# Autodesk Inventor assembly: Drive Roller Assembly
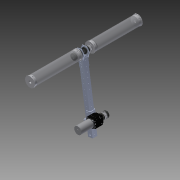
[picture p0: Inventor's stored thumbnail of the model, 180x180]
Saved by Autodesk Inventor 2014 SP1 (Build 180222100, 222)
## iProperties
Created: 2014-01-12
Part Number: Drive Roller Assembly
Document SubType Name: Assembly
Designer: Michael
Mass: 1125.53 g
Surface Area: 3756.72 cm^2
Volume: 516.176 cm^3
Density: 2.18052 g/cm^3
Author: Michael
## Documents named in this file (17)
- C:\Users\Arpan\Documents\GitHub\2014buildCAD\Collector\Drive Roller Assembly.iam
- C:\Users\Arpan\Documents\GitHub\2014buildCAD\Collector\Hex Shaft Collar 1-2 in (7552K500).ipt
- C:\Users\Arpan\Documents\GitHub\2014buildCAD\Collector\Timing Pulley (HTD 5mm) - 18T 9mm Double Flange, 1-2 in Hex (VexPro).ipt
- C:\Users\Arpan\Documents\GitHub\2014buildCAD\Collector\Hex Bearing 1-2 in (FR8ZZ-Hex, am-0279).ipt
- C:\Users\Arpan\Documents\GitHub\2014buildCAD\Collector\Hex Shaft 1-2 in (am-0856).ipt
- C:\Users\Arpan\Documents\GitHub\2014buildCAD\Collector\Roller End Cap Drive (3-D Printed).ipt
- C:\Users\Arpan\Documents\GitHub\2014buildCAD\Funnel Catcher\Vex Pro End Bearing Mount.ipt
- C:\Users\Arpan\Documents\GitHub\2014buildCAD\Funnel Catcher\Vex Pro 1x1 rectangular tubing 14 in length.ipt
- C:\Users\Arpan\Documents\GitHub\2014buildCAD\Collector\VersaPlanetary.iam
- C:\Users\Arpan\Documents\GitHub\2014buildCAD\Collector\Vex Pro VersaPlanetary Side Mount.ipt
- C:\Users\Arpan\Documents\GitHub\2014buildCAD\Collector\Polycarbonate Roller 2 OD 1-16 Thick (8585K64).ipt
- C:\Users\Arpan\Documents\GitHub\2014buildCAD\Collector\Drive Roller Assembly\AIP\FEA\axi0epmtc.fins
- C:\Users\Arpan\Documents\GitHub\2014buildCAD\Collector\Drive Roller Assembly\AIP\FEA\axi0epmu8.fsat
- C:\Users\Arpan\Documents\GitHub\2014buildCAD\Collector\Drive Roller Assembly\AIP\FEA\axi0epmu8.ftes
- C:\Users\Arpan\Documents\GitHub\2014buildCAD\Collector\Drive Roller Assembly\AIP\FEA\axi0epmu8.fwiz
- C:\Users\Arpan\Documents\GitHub\2014buildCAD\Collector\Drive Roller Assembly\AIP\FEA\axi0epnk0.fmsh
- C:\Users\Arpan\Documents\GitHub\2014buildCAD\Collector\Drive Roller Assembly\AIP\FEA\axi0epoao.fres
## Components (19 placed, 10 different names)
1. Timing Pulley (HTD 5mm) - 18T 9mm Double Flange, 1-2 in Hex (VexPro):1 — Mate:25, Mate:26, Mate:49, Mate:50
2. Hex Bearing 1-2 in (FR8ZZ-Hex, am-0279):1 — Insert:8, Mate:55, Mate:56, Mate:57
3. Hex Shaft Collar 1-2 in (7552K500):5 — Mate:31, Mate:32, Mate:50, Mate:55
4. Hex Shaft 1-2 in (am-0856):1 — Mate:25, Mate:26, Mate:31, Mate:32, Mate:33, Mate:34, Flush:1, Mate:56, Mate:57, Mate:59, Mate:60, Mate:62, Mate:63, Mate:84, Mate:85, Mate:88, Mate:89, Mate:91, Mate:92
5. Roller End Cap Drive (3-D Printed):1 — Mate:33, Mate:34, Flush:1, Mate:49, Insert:25, Mate:86, Mate:90
6. Vex Pro End Bearing Mount:1 — Insert:8, Mate:58, Insert:15, Insert:16
7. Hex Bearing 1-2 in (FR8ZZ-Hex, am-0279):2 — Insert:9, Mate:59, Mate:60, Mate:61
8. Hex Shaft Collar 1-2 in (7552K500):6 — Mate:61, Mate:62, Mate:63, Mate:83
9. Vex Pro End Bearing Mount:2 — Mate:58, Insert:9, Insert:13, Insert:14
10. Roller End Cap Drive (3-D Printed):2 — Insert:26, Mate:95
11. Vex Pro 1x1 rectangular tubing 14 in length:1 — Insert:13, Insert:14, Insert:15, Insert:16, Insert:23, Insert:24
12. VersaPlanetary:1 [sub-assembly] — Insert:21, Insert:22
13. Vex Pro VersaPlanetary Side Mount:1 — Insert:21, Insert:22, Insert:23, Insert:24
14. Roller End Cap Drive (3-D Printed):3 — Mate:83, Mate:84, Mate:85, Mate:87, Insert:28, Mate:93
15. Polycarbonate Roller 2 OD 1-16 Thick (8585K64):1 — Insert:25, Mate:86, Insert:26, Rotation:1, Mate:95
16. Roller End Cap Drive (3-D Printed):4 — Mate:94
17. Polycarbonate Roller 2 OD 1-16 Thick (8585K64):2 — Insert:28, Mate:93, Mate:94, Rotation:1
18. Hex Shaft Collar 1-2 in (7552K500):7 — Mate:87, Mate:88, Mate:89
19. Hex Shaft Collar 1-2 in (7552K500):8 — Mate:90, Mate:91, Mate:92
## Relationships (46: Mate 30, Insert 14, Flush 1, RelateRotation 1)
- Mate:25: Timing Pulley (HTD 5mm) - 18T 9mm Double Flange, 1-2 in Hex (VexPro):1 ↔ Hex Shaft 1-2 in (am-0856):1
- Mate:26: Timing Pulley (HTD 5mm) - 18T 9mm Double Flange, 1-2 in Hex (VexPro):1 ↔ Hex Shaft 1-2 in (am-0856):1
- Mate:31: Hex Shaft Collar 1-2 in (7552K500):5 ↔ Hex Shaft 1-2 in (am-0856):1
- Mate:32: Hex Shaft Collar 1-2 in (7552K500):5 ↔ Hex Shaft 1-2 in (am-0856):1
- Mate:33: Hex Shaft 1-2 in (am-0856):1 ↔ Roller End Cap Drive (3-D Printed):1
- Mate:34: Hex Shaft 1-2 in (am-0856):1 ↔ Roller End Cap Drive (3-D Printed):1
- Flush:1 (12.7 mm): Hex Shaft 1-2 in (am-0856):1 ↔ Roller End Cap Drive (3-D Printed):1
- Mate:49: Timing Pulley (HTD 5mm) - 18T 9mm Double Flange, 1-2 in Hex (VexPro):1 ↔ Roller End Cap Drive (3-D Printed):1
- Mate:50: Timing Pulley (HTD 5mm) - 18T 9mm Double Flange, 1-2 in Hex (VexPro):1 ↔ Hex Shaft Collar 1-2 in (7552K500):5
- Insert:8: Hex Bearing 1-2 in (FR8ZZ-Hex, am-0279):1 ↔ Vex Pro End Bearing Mount:1
- Mate:55: Hex Bearing 1-2 in (FR8ZZ-Hex, am-0279):1 ↔ Hex Shaft Collar 1-2 in (7552K500):5
- Mate:56: Hex Bearing 1-2 in (FR8ZZ-Hex, am-0279):1 ↔ Hex Shaft 1-2 in (am-0856):1
- Mate:57: Hex Bearing 1-2 in (FR8ZZ-Hex, am-0279):1 ↔ Hex Shaft 1-2 in (am-0856):1
- Mate:58 (25.4 mm): Vex Pro End Bearing Mount:1 ↔ Vex Pro End Bearing Mount:2
- Insert:9: Hex Bearing 1-2 in (FR8ZZ-Hex, am-0279):2 ↔ Vex Pro End Bearing Mount:2
- Mate:59: Hex Shaft 1-2 in (am-0856):1 ↔ Hex Bearing 1-2 in (FR8ZZ-Hex, am-0279):2
- Mate:60: Hex Shaft 1-2 in (am-0856):1 ↔ Hex Bearing 1-2 in (FR8ZZ-Hex, am-0279):2
- Mate:61: Hex Bearing 1-2 in (FR8ZZ-Hex, am-0279):2 ↔ Hex Shaft Collar 1-2 in (7552K500):6
- Mate:62: Hex Shaft 1-2 in (am-0856):1 ↔ Hex Shaft Collar 1-2 in (7552K500):6
- Mate:63: Hex Shaft 1-2 in (am-0856):1 ↔ Hex Shaft Collar 1-2 in (7552K500):6
- Insert:13: Vex Pro End Bearing Mount:2 ↔ Vex Pro 1x1 rectangular tubing 14 in length:1
- Insert:14: Vex Pro End Bearing Mount:2 ↔ Vex Pro 1x1 rectangular tubing 14 in length:1
- Insert:15: Vex Pro End Bearing Mount:1 ↔ Vex Pro 1x1 rectangular tubing 14 in length:1
- Insert:16: Vex Pro End Bearing Mount:1 ↔ Vex Pro 1x1 rectangular tubing 14 in length:1
- Insert:21: VersaPlanetary:1 ↔ Vex Pro VersaPlanetary Side Mount:1
- Insert:22: VersaPlanetary:1 ↔ Vex Pro VersaPlanetary Side Mount:1
- Insert:23: Vex Pro 1x1 rectangular tubing 14 in length:1 ↔ Vex Pro VersaPlanetary Side Mount:1
- Insert:24: Vex Pro 1x1 rectangular tubing 14 in length:1 ↔ Vex Pro VersaPlanetary Side Mount:1
- Mate:83: Hex Shaft Collar 1-2 in (7552K500):6 ↔ Roller End Cap Drive (3-D Printed):3
- Mate:84: Hex Shaft 1-2 in (am-0856):1 ↔ Roller End Cap Drive (3-D Printed):3
- Mate:85: Hex Shaft 1-2 in (am-0856):1 ↔ Roller End Cap Drive (3-D Printed):3
- Insert:25: Roller End Cap Drive (3-D Printed):1 ↔ Polycarbonate Roller 2 OD 1-16 Thick (8585K64):1
- Mate:86: Roller End Cap Drive (3-D Printed):1 ↔ Polycarbonate Roller 2 OD 1-16 Thick (8585K64):1
- Insert:26: Roller End Cap Drive (3-D Printed):2 ↔ Polycarbonate Roller 2 OD 1-16 Thick (8585K64):1
- [Insert]: Roller End Cap Drive (3-D Printed):4 ↔ Polycarbonate Roller 2 OD 1-16 Thick (8585K64):2
- Mate:87: Roller End Cap Drive (3-D Printed):3 ↔ Hex Shaft Collar 1-2 in (7552K500):7
- Mate:88: Hex Shaft 1-2 in (am-0856):1 ↔ Hex Shaft Collar 1-2 in (7552K500):7
- Mate:89: Hex Shaft 1-2 in (am-0856):1 ↔ Hex Shaft Collar 1-2 in (7552K500):7
- Mate:90: Roller End Cap Drive (3-D Printed):1 ↔ Hex Shaft Collar 1-2 in (7552K500):8
- Mate:91: Hex Shaft 1-2 in (am-0856):1 ↔ Hex Shaft Collar 1-2 in (7552K500):8
- Mate:92: Hex Shaft 1-2 in (am-0856):1 ↔ Hex Shaft Collar 1-2 in (7552K500):8
- Insert:28: Roller End Cap Drive (3-D Printed):3 ↔ Polycarbonate Roller 2 OD 1-16 Thick (8585K64):2
- Mate:93: Roller End Cap Drive (3-D Printed):3 ↔ Polycarbonate Roller 2 OD 1-16 Thick (8585K64):2
- Mate:94: Roller End Cap Drive (3-D Printed):4 ↔ Polycarbonate Roller 2 OD 1-16 Thick (8585K64):2
- Rotation:1 [RelateRotation] (1 ul): Polycarbonate Roller 2 OD 1-16 Thick (8585K64):1 ↔ Polycarbonate Roller 2 OD 1-16 Thick (8585K64):2
- Mate:95: Roller End Cap Drive (3-D Printed):2 ↔ Polycarbonate Roller 2 OD 1-16 Thick (8585K64):1
## Named parameters: sa_0 = -444.138, sa_1 = 24.6654, sa_2 = 0, d138_d137 = 0 mm, sa_3 = 8896.44
note: some values were not read from the file. Shown as the stored number, unit unknown: "sa_0", "sa_1", "sa_2", "sa_3".
